# Autodesk Inventor assembly: Prototipo Inicial
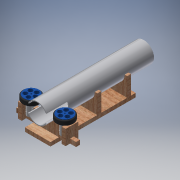
[picture p0: Inventor's stored thumbnail of the model, 180x180]
Saved by Autodesk Inventor 2016 SP2 (Build 200236200, 236)
## iProperties
Created: 2017-06-26
Part Number: Prototipo Inicial
Material: Genérico
Document SubType Name: Assembly
Designer: ssant
Author: ssant
## Documents named in this file (8)
- C:\Users\ssant\Documents\My Works\Trabajos Varios\Proyectos\VirPong\CAD\Prototipo Inicial.iam
- C:\Users\ssant\Documents\My Works\Trabajos Varios\Proyectos\VirPong\CAD\Base Prototipo Inicial.ipt
- C:\Users\ssant\Documents\My Works\Trabajos Varios\Proyectos\VirPong\CAD\Soporte para Motor Prototipo Inicial.ipt
- C:\Users\ssant\Documents\My Works\Trabajos Varios\Proyectos\VirPong\CAD\Soporte para Cañón Prototio Inicial.ipt
- C:\Users\ssant\Documents\My Works\Trabajos Varios\Proyectos\VirPong\CAD\Cañón Prototipo Inicial.ipt
- C:\Users\ssant\Documents\My Works\Trabajos Varios\Proyectos\VirPong\CAD\Motor Prototipo Inicial.ipt
- C:\Users\ssant\Documents\My Works\Trabajos Varios\Proyectos\VirPong\CAD\Rueda Prototipo Inicial.ipt
- C:\Users\ssant\Documents\My Works\Trabajos Varios\Proyectos\VirPong\CAD\Tope para Motor Prototipo Inicial.ipt
## Components (11 placed, 7 different names)
1. Base Prototipo Inicial:1 — Coincidencia:1, Nivelación:1, Nivelación:2, Coincidencia:2, Coincidencia:3, Nivelación:3, Nivelación:4, Nivelación:5
2. Soporte para Motor Prototipo Inicial:1 — Coincidencia:1, Nivelación:1, Nivelación:2, Coincidencia:6, Coincidencia:7, Nivelación:8, Coincidencia:10, Coincidencia:11, Coincidencia:12, Nivelación:13, Coincidencia:13
3. Soporte para Cañón Prototio Inicial:1 — Coincidencia:2, Nivelación:3, Nivelación:5, Nivelación:6, Rígido:1
4. Soporte para Cañón Prototio Inicial:2 — Coincidencia:3, Nivelación:4, Nivelación:6
5. Motor Prototipo Inicial:1 — Insertar:1, Coincidencia:8, Nivelación:9, Nivelación:12, Coincidencia:10
6. Motor Prototipo Inicial:2 — Insertar:2, Coincidencia:9, Nivelación:10, Nivelación:11, Coincidencia:13
7. Rueda Prototipo Inicial:1 — Insertar:2
8. Rueda Prototipo Inicial:2 — Insertar:1
9. Tope para Motor Prototipo Inicial:1 — Coincidencia:9, Nivelación:10, Nivelación:11, Coincidencia:11, Coincidencia:12, Nivelación:13
10. Tope para Motor Prototipo Inicial:2 — Coincidencia:6, Coincidencia:7, Nivelación:8, Coincidencia:8, Nivelación:9, Nivelación:12
11. Cañón Prototipo Inicial:1 — Rígido:1
## Relationships (26: Flush 12, Mate 11, Insert 2, WeldJoint 1)
- Coincidencia:1 [Mate]: Base Prototipo Inicial:1 ↔ Soporte para Motor Prototipo Inicial:1
- Nivelación:1 [Flush]: Base Prototipo Inicial:1 ↔ Soporte para Motor Prototipo Inicial:1
- Nivelación:2 [Flush] (20 mm): Base Prototipo Inicial:1 ↔ Soporte para Motor Prototipo Inicial:1
- Coincidencia:2 [Mate]: Base Prototipo Inicial:1 ↔ Soporte para Cañón Prototio Inicial:1
- Coincidencia:3 [Mate]: Base Prototipo Inicial:1 ↔ Soporte para Cañón Prototio Inicial:2
- Nivelación:3 [Flush]: Base Prototipo Inicial:1 ↔ Soporte para Cañón Prototio Inicial:1
- Nivelación:4 [Flush]: Base Prototipo Inicial:1 ↔ Soporte para Cañón Prototio Inicial:2
- Nivelación:5 [Flush] (110 mm): Base Prototipo Inicial:1 ↔ Soporte para Cañón Prototio Inicial:1
- Nivelación:6 [Flush] (70 mm): Soporte para Cañón Prototio Inicial:1 ↔ Soporte para Cañón Prototio Inicial:2
- Insertar:1: Motor Prototipo Inicial:1 ↔ Rueda Prototipo Inicial:2
- Insertar:2: Motor Prototipo Inicial:2 ↔ Rueda Prototipo Inicial:1
- Coincidencia:6 [Mate]: Soporte para Motor Prototipo Inicial:1 ↔ Tope para Motor Prototipo Inicial:2
- Coincidencia:7 [Mate]: Soporte para Motor Prototipo Inicial:1 ↔ Tope para Motor Prototipo Inicial:2
- Nivelación:8 [Flush]: Soporte para Motor Prototipo Inicial:1 ↔ Tope para Motor Prototipo Inicial:2
- Coincidencia:8 [Mate]: Motor Prototipo Inicial:1 ↔ Tope para Motor Prototipo Inicial:2
- Nivelación:9 [Flush]: Motor Prototipo Inicial:1 ↔ Tope para Motor Prototipo Inicial:2
- Coincidencia:9 [Mate]: Motor Prototipo Inicial:2 ↔ Tope para Motor Prototipo Inicial:1
- Nivelación:10 [Flush]: Motor Prototipo Inicial:2 ↔ Tope para Motor Prototipo Inicial:1
- Nivelación:11 [Flush] (-2.5 mm): Motor Prototipo Inicial:2 ↔ Tope para Motor Prototipo Inicial:1
- Nivelación:12 [Flush] (-2.5 mm): Motor Prototipo Inicial:1 ↔ Tope para Motor Prototipo Inicial:2
- Coincidencia:10 [Mate] (2 mm): Soporte para Motor Prototipo Inicial:1 ↔ Motor Prototipo Inicial:1
- Coincidencia:11 [Mate]: Soporte para Motor Prototipo Inicial:1 ↔ Tope para Motor Prototipo Inicial:1
- Coincidencia:12 [Mate]: Soporte para Motor Prototipo Inicial:1 ↔ Tope para Motor Prototipo Inicial:1
- Nivelación:13 [Flush]: Soporte para Motor Prototipo Inicial:1 ↔ Tope para Motor Prototipo Inicial:1
- Coincidencia:13 [Mate] (2 mm): Soporte para Motor Prototipo Inicial:1 ↔ Motor Prototipo Inicial:2
- Rígido:1 [WeldJoint] (-5 mm): Soporte para Cañón Prototio Inicial:1 ↔ Cañón Prototipo Inicial:1
